# Autodesk Inventor assembly: CS2Mazebot
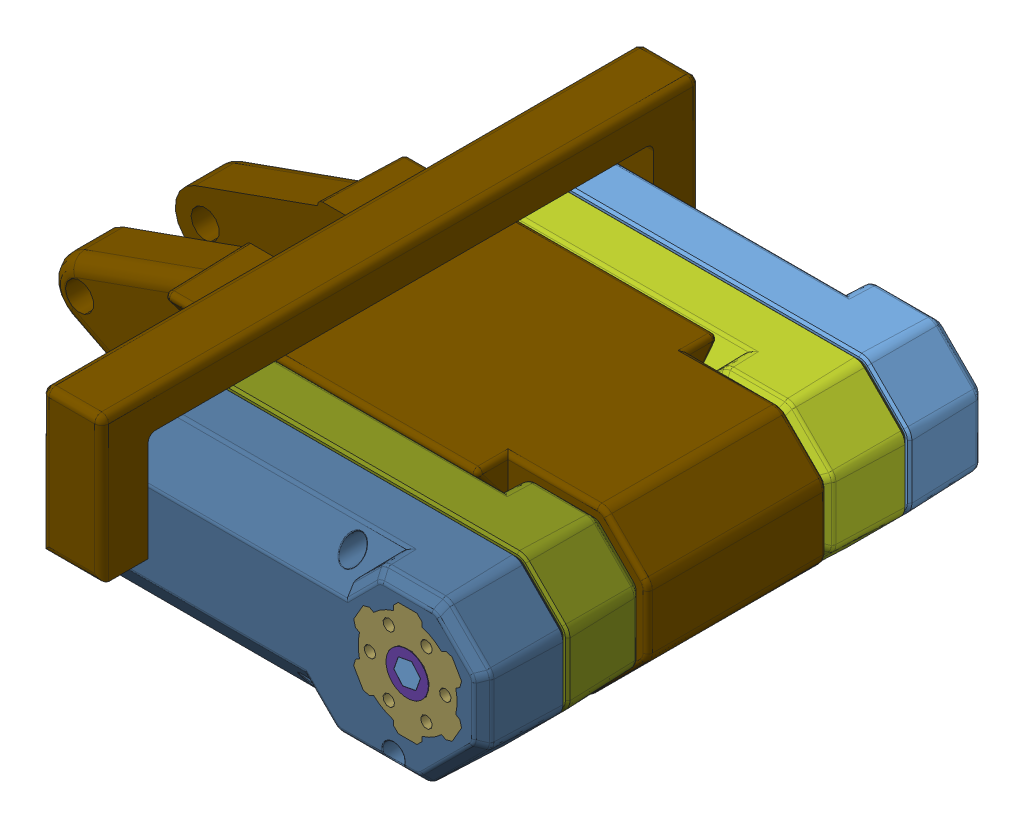
[picture p0: shaded view drawn from the shape stored in the file]
Saved by Autodesk Inventor 2018 (Build 220112000, 112)
## iProperties
Created: 2018-04-18
Part Number: CS2Mazebot
Document SubType Name: Assembly
Designer: Samuel
Author: Samuel
## Documents named in this file (5)
- C:\Users\Samuel Schuur\Documents\CS2\CS2Mazebot.iam
- C:\Users\Samuel Schuur\Downloads\REV-41-1300.ipt
- C:\Users\Samuel Schuur\Downloads\REV-41-1300_MIR.ipt
- C:\Users\Samuel Schuur\Documents\CS2\ChassisBase.ipt
- C:\Users\Samuel Schuur\Documents\Shaft.ipt
## Components (4 placed, 4 different names)
1. REV-41-1300:1 — Flush:1, Flush:2
2. REV-41-1300_MIR:1 — Mate:1, Flush:3
3. ChassisBase:1 — Flush:2
4. Shaft:1 — Flush:3
## Relationships (4: Flush 3, Mate 1)
- Flush:1 (19.05 mm): REV-41-1300:1
- Mate:1 (19.05 mm): REV-41-1300_MIR:1
- Flush:2: REV-41-1300:1 ↔ ChassisBase:1
- Flush:3: REV-41-1300_MIR:1 ↔ Shaft:1
